# Autodesk Inventor assembly: Assembly1
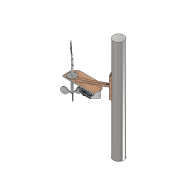
[picture p0: Inventor's stored thumbnail of the model, 180x180]
Saved by Autodesk Inventor 2022 (Build 260153000, 153)
## iProperties
Created: 2025-07-11
Part Number: Assembly1
Document SubType Name: Assembly
Designer: 1234
Author: 1234
## Documents named in this file (21)
- C:\Users\sacchie\Dropbox\Giorgio_Mac\PPS (pascon piccone sacchiero)\componenti\Assembly1.iam
- C:\Users\sacchie\Dropbox\Giorgio_Mac\PPS (pascon piccone sacchiero)\componenti\pannello solare.ipt
- C:\Users\sacchie\Dropbox\Giorgio_Mac\PPS (pascon piccone sacchiero)\componenti\scatola corpo.ipt
- C:\Users\sacchie\Dropbox\Giorgio_Mac\PPS (pascon piccone sacchiero)\componenti\sacatola coperchio principale.ipt
- C:\Users\sacchie\Dropbox\Giorgio_Mac\PPS (pascon piccone sacchiero)\componenti\Tower Pro MG996R.ipt
- C:\Users\sacchie\Dropbox\Giorgio_Mac\PPS (pascon piccone sacchiero)\componenti\guarnizione motore.ipt
- C:\Users\sacchie\Dropbox\Giorgio_Mac\PPS (pascon piccone sacchiero)\componenti\adattatore per motore.ipt
- C:\Users\sacchie\Dropbox\Giorgio_Mac\PPS (pascon piccone sacchiero)\componenti\cupola alta di protezione.ipt
- C:\Users\sacchie\Dropbox\Giorgio_Mac\PPS (pascon piccone sacchiero)\componenti\manometro idealmente.ipt
- C:\Users\sacchie\Dropbox\Giorgio_Mac\PPS (pascon piccone sacchiero)\componenti\legno.ipt
- C:\Users\sacchie\Dropbox\Giorgio_Mac\PPS (pascon piccone sacchiero)\componenti\direzione del vento.ipt
- C:\Users\sacchie\Dropbox\Giorgio_Mac\PPS (pascon piccone sacchiero)\componenti\legno 1.ipt
- C:\Users\sacchie\Dropbox\Giorgio_Mac\PPS (pascon piccone sacchiero)\componenti\legno 2.ipt
- C:\Users\sacchie\Dropbox\Giorgio_Mac\PPS (pascon piccone sacchiero)\componenti\profiletto a l.ipt
- C:\Users\sacchie\Dropbox\Giorgio_Mac\PPS (pascon piccone sacchiero)\componenti\lampione.ipt
- C:\Users\sacchie\Dropbox\Giorgio_Mac\PPS (pascon piccone sacchiero)\componenti\spazzola - asta.ipt
- C:\Users\sacchie\Dropbox\Giorgio_Mac\PPS (pascon piccone sacchiero)\componenti\spazzola - spazzola.ipt
- C:\Users\sacchie\Dropbox\Giorgio_Mac\PPS (pascon piccone sacchiero)\componenti\spessori.ipt
- C:\Users\sacchie\Dropbox\Giorgio_Mac\PPS (pascon piccone sacchiero)\componenti\PPS_pcb_v1.ipt
- C:\Users\sacchie\Dropbox\Giorgio_Mac\PPS (pascon piccone sacchiero)\componenti\piedino.ipt
- C:\Users\sacchie\Dropbox\Giorgio_Mac\PPS (pascon piccone sacchiero)\componenti\tappino tpu.ipt
## Components (27 placed, 20 different names)
1. scatola corpo:1 — Mate:9, Mate:10, Mate:11, Mate:18, Mate:29, Mate:30, Mate:31, Mate:39, Mate:40, Mate:45, Mate:46, Flush:5, Mate:68, Mate:101, Mate:102
2. sacatola coperchio principale:1 — Mate:9, Mate:10, Mate:11, Mate:47, Mate:49, Mate:86, Mate:93, Angle:3, Mate:94, Mate:97, Mate:98, Mate:99, Mate:100, Mate:103
3. pannello solare:2 — Mate:18, Flush:5, Mate:68
4. Tower Pro MG996R:1 — Mate:29, Mate:30, Mate:35, Mate:36, Mate:43, Mate:44, Mate:45
5. guarnizione motore:2 — Mate:31, Mate:43, Mate:44
6. adattatore per motore:2 — Mate:35, Mate:36, Mate:73, Mate:74, Mate:75
7. cupola alta di protezione:1 — Mate:39, Mate:40, Mate:46
8. legno:1 — Mate:47, Mate:49, Mate:50, Mate:54, Flush:1, Flush:2, Mate:55, Mate:56, Mate:57, Mate:64, Mate:66, Mate:78, Mate:79, Mate:80, Mate:81, Mate:82, Mate:83, Mate:84, Mate:85
9. manometro idealmente:1 — Mate:50, Mate:66, Mate:67
10. direzione del vento:1 — Mate:64, Mate:67
11. legno 1:1 — Mate:55, Mate:56, Mate:57, Mate:62, Mate:63, Flush:3, Flush:4, Mate:87, Mate:88
12. legno 2:1 — Mate:87, Mate:88, Mate:89, Mate:90, Angle:2, Mate:91
13. profiletto a l:1 — Mate:62, Flush:4, Mate:90
14. profiletto a l:2 — Mate:63, Flush:3, Mate:89
15. lampione:1 — Angle:1, Angle:2, Mate:91
16. spazzola - asta:1 — Mate:73, Mate:74, Mate:75, Mate:76, Mate:77, Flush:6
17. spazzola - spazzola:1 — Mate:76, Mate:77, Flush:6
18. spessori:1 — Mate:82, Mate:83
19. spessori:2 — Mate:81, Mate:84
20. spessori:3 — Mate:80, Mate:85, Mate:86
21. spessori:4 — Mate:78, Mate:79
22. PPS_pcb_v1:1 — Mate:93, Angle:3, Mate:96
23. piedino:2 — Mate:97, Mate:98
24. piedino:3 — Mate:94, Mate:96, Mate:103
25. piedino:4 — Mate:99, Mate:100
26. tappino tpu:1
27. tappino tpu:2 — Mate:101, Mate:102
## Relationships (66: Mate 57, Flush 6, Angle 3)
- Mate:9: scatola corpo:1 ↔ sacatola coperchio principale:1
- Mate:10: scatola corpo:1 ↔ sacatola coperchio principale:1
- Mate:11: scatola corpo:1 ↔ sacatola coperchio principale:1
- Mate:18: scatola corpo:1 ↔ pannello solare:2
- Mate:29: scatola corpo:1 ↔ Tower Pro MG996R:1
- Mate:30: scatola corpo:1 ↔ Tower Pro MG996R:1
- Mate:31: scatola corpo:1 ↔ guarnizione motore:2
- Mate:35: Tower Pro MG996R:1 ↔ adattatore per motore:2
- Mate:36 (0.5 mm): Tower Pro MG996R:1 ↔ adattatore per motore:2
- Mate:39: scatola corpo:1 ↔ cupola alta di protezione:1
- Mate:40: scatola corpo:1 ↔ cupola alta di protezione:1
- Mate:43: Tower Pro MG996R:1 ↔ guarnizione motore:2
- Mate:44: Tower Pro MG996R:1 ↔ guarnizione motore:2
- Mate:45: scatola corpo:1 ↔ Tower Pro MG996R:1
- Mate:46: scatola corpo:1 ↔ cupola alta di protezione:1
- Mate:47: sacatola coperchio principale:1 ↔ legno:1
- Mate:49: sacatola coperchio principale:1 ↔ legno:1
- Mate:50: legno:1 ↔ manometro idealmente:1
- Mate:54: legno:1
- Flush:1: legno:1
- Flush:2: legno:1
- Mate:55: legno:1 ↔ legno 1:1
- Mate:56: legno:1 ↔ legno 1:1
- Mate:57: legno:1 ↔ legno 1:1
- Mate:62: legno 1:1 ↔ profiletto a l:1
- Mate:63: legno 1:1 ↔ profiletto a l:2
- Flush:3 (5 mm): legno 1:1 ↔ profiletto a l:2
- Flush:4 (5 mm): legno 1:1 ↔ profiletto a l:1
- Mate:64: legno:1 ↔ direzione del vento:1
- Mate:66: legno:1 ↔ manometro idealmente:1
- Mate:67: manometro idealmente:1 ↔ direzione del vento:1
- Flush:5 (13 mm): scatola corpo:1 ↔ pannello solare:2
- Mate:68 (4 mm): scatola corpo:1 ↔ pannello solare:2
- Mate:73: adattatore per motore:2 ↔ spazzola - asta:1
- Mate:74: adattatore per motore:2 ↔ spazzola - asta:1
- Mate:75: adattatore per motore:2 ↔ spazzola - asta:1
- Mate:76 (0.1 mm): spazzola - asta:1 ↔ spazzola - spazzola:1
- Mate:77 (0.1 mm): spazzola - asta:1 ↔ spazzola - spazzola:1
- Flush:6: spazzola - asta:1 ↔ spazzola - spazzola:1
- Mate:78: legno:1 ↔ spessori:4
- Mate:79: legno:1 ↔ spessori:4
- Mate:80: legno:1 ↔ spessori:3
- Mate:81: legno:1 ↔ spessori:2
- Mate:82: legno:1 ↔ spessori:1
- Mate:83: legno:1 ↔ spessori:1
- Mate:84: legno:1 ↔ spessori:2
- Mate:85: legno:1 ↔ spessori:3
- Mate:86: sacatola coperchio principale:1 ↔ spessori:3
- Mate:87: legno 1:1 ↔ legno 2:1
- Mate:88: legno 1:1 ↔ legno 2:1
- Mate:89: legno 2:1 ↔ profiletto a l:2
- Mate:90: legno 2:1 ↔ profiletto a l:1
- Angle:1 (0 deg): lampione:1
- Angle:2 (0 deg): legno 2:1 ↔ lampione:1
- Mate:91: legno 2:1 ↔ lampione:1
- Mate:93: sacatola coperchio principale:1 ↔ PPS_pcb_v1:1
- Angle:3 (0 deg): sacatola coperchio principale:1 ↔ PPS_pcb_v1:1
- Mate:94: sacatola coperchio principale:1 ↔ piedino:3
- Mate:96: PPS_pcb_v1:1 ↔ piedino:3
- Mate:97: sacatola coperchio principale:1 ↔ piedino:2
- Mate:98: sacatola coperchio principale:1 ↔ piedino:2
- Mate:99: sacatola coperchio principale:1 ↔ piedino:4
- Mate:100: sacatola coperchio principale:1 ↔ piedino:4
- Mate:101: scatola corpo:1 ↔ tappino tpu:2
- Mate:102: scatola corpo:1 ↔ tappino tpu:2
- Mate:103: sacatola coperchio principale:1 ↔ piedino:3
